# Autodesk Inventor assembly: Toughbox Mini L-Base
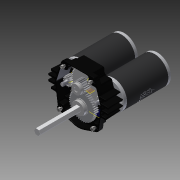
[picture p0: Inventor's stored thumbnail of the model, 180x180]
Saved by Autodesk Inventor 2015 SP1 (Build 190203100, 203)
## iProperties
Created: 2014-12-16
Part Number: Toughbox Mini L-Base
Document SubType Name: Assembly
Designer: Philip
Author: Philip
## Documents named in this file (17)
- D:\Data Folder\FIRST 2015\KOP_FRC\Drive Base\Parts\Toughbox Mini L-Base.iam
- D:\Data Folder\FIRST 2015\KOP_FRC\Drive Base\Parts\TB Output Shaft Hex L-Base 2.ipt
- D:\Data Folder\FIRST 2015\KOP_FRC\Drive Base\Parts\Toughbox d07.ipt
- D:\Data Folder\FIRST 2015\KOP_FRC\Drive Base\Parts\Toughbox d05.ipt
- D:\Data Folder\FIRST 2015\KOP_FRC\Drive Base\Parts\10-32 Nylock Nut.ipt
- D:\Data Folder\FIRST 2015\KOP_FRC\Drive Base\Parts\5-16 washer.ipt
- D:\Data Folder\FIRST 2015\KOP_FRC\Drive Base\Parts\Toughbox d09.ipt
- D:\Data Folder\FIRST 2015\KOP_FRC\Drive Base\Parts\TM Housing.ipt
- D:\Data Folder\FIRST 2015\KOP_FRC\Drive Base\Parts\SHCS 10-32 x 0.625.ipt
- D:\Data Folder\FIRST 2015\KOP_FRC\Drive Base\Parts\R6ZZ Bearing.ipt
- D:\Data Folder\FIRST 2015\KOP_FRC\Drive Base\Parts\8mm spring clip.ipt
- D:\Data Folder\FIRST 2015\KOP_FRC\Drive Base\Parts\500 E-klip.ipt
- D:\Data Folder\FIRST 2015\KOP_FRC\Drive Base\Parts\FR8ZZ Hex Bearing.ipt
- D:\Data Folder\FIRST 2015\KOP_FRC\Drive Base\Parts\FR6ZZ Bearing.ipt
- D:\Data Folder\FIRST 2015\KOP_FRC\Drive Base\Parts\45T 20dp 500h_Inch - Spur gear 20DP 45T 14.5PA .4FW ---S45N.5H1L0.5N.ipt
- D:\Data Folder\FIRST 2015\KOP_FRC\Drive Base\Parts\19T 20dp 375h_Inch - Spur gear 20DP 19T 14.5PA .575FW ---S19N.5H1L0.375N.ipt
- D:\Data Folder\FIRST 2015\KOP_FRC\Drive Base\Parts\MOT_CIM-Motor_217-2000.iam
## Components (33 placed, 33 different names)
1. TB Output Shaft Hex L-Base 2_57 — Mate:23, Mate:24, Angle:1, Mate:27
2. Toughbox d07_58 — Mate:6, Mate:10, Mate:25, Mate:26
3. Toughbox d05_59 — Mate:5, Mate:6, Mate:7, Mate:8, Mate:9, Mate:13, Mate:16, Rotation:1, Rotation:2
4. 10-32 Nylock Nut_60
5. 10-32 Nylock Nut_61
6. 10-32 Nylock Nut_62
7. 10-32 Nylock Nut_63
8. 5-16 washer_64
9. 5-16 washer_65 — Mate:15
10. 5-16 washer_66 — Mate:12
11. 5-16 washer_67
12. Toughbox d09_68 — Mate:14, Mate:15, Mate:16, Rotation:2
13. Toughbox d09_69 — Mate:11, Mate:12, Mate:13, Rotation:1
14. TM Housing_70 — Insert:1, Mate:4, Mate:21, Mate:22, Mate:24
15. SHCS 10-32 x 0.625_71 — Mate:1
16. SHCS 10-32 x 0.625_72
17. SHCS 10-32 x 0.625_73
18. SHCS 10-32 x 0.625_74
19. SHCS 10-32 x 0.625_75
20. SHCS 10-32 x 0.625_76
21. SHCS 10-32 x 0.625_77 — Mate:2
22. SHCS 10-32 x 0.625_78 — Mate:3
23. R6ZZ Bearing_79 — Mate:5, Mate:7, Mate:25, Mate:26
24. R6ZZ Bearing_80 — Mate:21, Mate:22, Mate:23, Mate:28
25. 8mm spring clip_81
26. 8mm spring clip_82
27. 500 E-klip_83
28. FR8ZZ Hex Bearing_84 — Mate:17, Mate:18, Mate:19, Mate:27
29. FR6ZZ Bearing_85
30. CIM Motor SW_86 [sub-assembly] — Insert:1, Mate:1, Mate:14
31. CIM Motor SW_87 [sub-assembly] — Mate:2, Mate:3, Mate:4, Mate:11
32. 45T 20dp 500h_Inch - Spur gear 20DP 45T 14.5PA .4FW ---S45N.5H1L0.5N_88 — Mate:18, Mate:19, Angle:1, Angle:2, Rotation:3, Mate:28
33. 19T 20dp 375h_Inch - Spur gear 20DP 19T 14.5PA .575FW ---S19N.5H1L0.375N_89 — Mate:8, Mate:9, Mate:10, Angle:2, Rotation:3
## Relationships (33: Mate 27, RelateRotation 3, Angle 2, Insert 1)
- Insert:1: TM Housing_70 ↔ CIM Motor SW_86
- Mate:1: SHCS 10-32 x 0.625_71 ↔ CIM Motor SW_86
- Mate:2: SHCS 10-32 x 0.625_77 ↔ CIM Motor SW_87
- Mate:3: SHCS 10-32 x 0.625_78 ↔ CIM Motor SW_87
- Mate:4: TM Housing_70 ↔ CIM Motor SW_87
- Mate:5: Toughbox d05_59 ↔ R6ZZ Bearing_79
- Mate:6: Toughbox d07_58 ↔ Toughbox d05_59
- Mate:7: Toughbox d05_59 ↔ R6ZZ Bearing_79
- Mate:8: Toughbox d05_59 ↔ 19T 20dp 375h_Inch - Spur gear 20DP 19T 14.5PA .575FW ---S19N.5H1L0.375N_89
- Mate:9: Toughbox d05_59 ↔ 19T 20dp 375h_Inch - Spur gear 20DP 19T 14.5PA .575FW ---S19N.5H1L0.375N_89
- Mate:10: Toughbox d07_58 ↔ 19T 20dp 375h_Inch - Spur gear 20DP 19T 14.5PA .575FW ---S19N.5H1L0.375N_89
- Mate:11: Toughbox d09_69 ↔ CIM Motor SW_87
- Mate:12: 5-16 washer_66 ↔ Toughbox d09_69
- Mate:13: Toughbox d05_59 ↔ Toughbox d09_69
- Mate:14: Toughbox d09_68 ↔ CIM Motor SW_86
- Mate:15: 5-16 washer_65 ↔ Toughbox d09_68
- Mate:16: Toughbox d05_59 ↔ Toughbox d09_68
- Mate:17: FR8ZZ Hex Bearing_84
- Mate:18: FR8ZZ Hex Bearing_84 ↔ 45T 20dp 500h_Inch - Spur gear 20DP 45T 14.5PA .4FW ---S45N.5H1L0.5N_88
- Mate:19: FR8ZZ Hex Bearing_84 ↔ 45T 20dp 500h_Inch - Spur gear 20DP 45T 14.5PA .4FW ---S45N.5H1L0.5N_88
- Mate:21: TM Housing_70 ↔ R6ZZ Bearing_80
- Mate:22: TM Housing_70 ↔ R6ZZ Bearing_80
- Mate:23: TB Output Shaft Hex L-Base 2_57 ↔ R6ZZ Bearing_80
- Mate:24: TB Output Shaft Hex L-Base 2_57 ↔ TM Housing_70
- Angle:1 (0 deg): TB Output Shaft Hex L-Base 2_57 ↔ 45T 20dp 500h_Inch - Spur gear 20DP 45T 14.5PA .4FW ---S45N.5H1L0.5N_88
- Angle:2 (0 deg): 45T 20dp 500h_Inch - Spur gear 20DP 45T 14.5PA .4FW ---S45N.5H1L0.5N_88 ↔ 19T 20dp 375h_Inch - Spur gear 20DP 19T 14.5PA .575FW ---S19N.5H1L0.375N_89
- Rotation:1 [RelateRotation] (0.3077 ul): Toughbox d05_59 ↔ Toughbox d09_69
- Rotation:2 [RelateRotation] (0.4038 ul): Toughbox d05_59 ↔ Toughbox d09_68
- Rotation:3 [RelateRotation] (0.4038 ul): 45T 20dp 500h_Inch - Spur gear 20DP 45T 14.5PA .4FW ---S45N.5H1L0.5N_88 ↔ 19T 20dp 375h_Inch - Spur gear 20DP 19T 14.5PA .575FW ---S19N.5H1L0.375N_89
- Mate:25: Toughbox d07_58 ↔ R6ZZ Bearing_79
- Mate:26: Toughbox d07_58 ↔ R6ZZ Bearing_79
- Mate:27: TB Output Shaft Hex L-Base 2_57 ↔ FR8ZZ Hex Bearing_84
- Mate:28: R6ZZ Bearing_80 ↔ 45T 20dp 500h_Inch - Spur gear 20DP 45T 14.5PA .4FW ---S45N.5H1L0.5N_88
